# Autodesk Inventor assembly: Assembly1
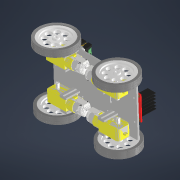
[picture p0: Inventor's stored thumbnail of the model, 180x180]
Saved by Autodesk Inventor 2021 (Build 250183000, 183)
## iProperties
Created: 2022-06-26
Part Number: Assembly1
Document SubType Name: Assembly
Designer: phand
Author: phand
## Documents named in this file (9)
- D:\Kien Phan\University\Training\Bluetooth controlling car\3D\Assembly1.iam
- D:\Kien Phan\University\Training\Bluetooth controlling car\3D\chassis.ipt
- D:\Kien Phan\University\Training\Bluetooth controlling car\3D\Ga motor 1.ipt
- D:\Kien Phan\University\Training\Bluetooth controlling car\3D\YG2900_step.ipt
- D:\Kien Phan\University\IAC Club\Animal Robot\Line follower robot\v4\rubber-wheel-65mm-1.snapshot.1\Whell - 65mm\Llanta.ipt
- D:\Kien Phan\University\IAC Club\Animal Robot\Line follower robot\v4\l298n-stepper-motor-driver-red-1.snapshot.3\L298N Stepper Motor Driver (Red).ipt
- D:\Kien Phan\University\Training\Bluetooth controlling car\3D\18650 battery holder part.ipt
- D:\Kien Phan\University\Training\Bluetooth controlling car\3D\mid chassis.ipt
- D:\Kien Phan\Inventor Library\Parts\Arduino Uno.ipt
## Components (21 placed, 8 different names)
1. chassis:1 — Mate:1, Mate:2, Mate:4, Mate:6, Mate:7, Mate:8, Mate:9, Mate:10, Mate:11, Mate:12, Mate:15, Mate:16, Mate:17, Mate:22, Mate:23, Mate:24, Mate:25, Mate:26, Mate:27, Mate:30, Mate:31, Mate:32, Mate:33, Mate:34, Mate:35, Mate:38, Mate:45, Mate:46, Mate:48, Mate:50, Mate:53, Mate:54, Mate:55
2. YG2900_step:4 — Mate:36, Mate:37, Mate:42
3. Ga motor 1:1 — Mate:1, Mate:2, Mate:4, Mate:6, Mate:21, Mate:38
4. Ga motor 1:2 — Mate:7, Mate:8, Mate:9, Mate:20
5. Ga motor 1:3 — Mate:15, Mate:16, Mate:17
6. Ga motor 1:4 — Mate:10, Mate:11, Mate:12, Mate:18, Mate:19
7. Ga motor 1:5 — Mate:32, Mate:33, Mate:34, Mate:36, Mate:37
8. Ga motor 1:6 — Mate:30, Mate:31, Mate:35, Mate:48
9. Ga motor 1:7 — Mate:25, Mate:26, Mate:27
10. Ga motor 1:8 — Mate:22, Mate:23, Mate:24, Mate:28, Mate:29
11. YG2900_step:5 — Mate:20, Mate:21, Mate:39
12. YG2900_step:6 — Mate:18, Mate:19, Mate:41
13. YG2900_step:7 — Mate:28, Mate:29, Mate:43
14. Llanta:1 — Mate:39
15. Llanta:3 — Mate:41
16. Llanta:4 — Mate:43
17. Llanta:5 — Mate:42
18. L298N Stepper Motor Driver (Red):1 — Mate:45, Mate:46
19. 18650 battery holder part:1 — Mate:52
20. mid chassis:1 — Mate:50, Mate:52
21. Arduino Uno:1 — Mate:53, Mate:54, Mate:55
## Relationships (46: Mate 46)
- Mate:1: chassis:1 ↔ Ga motor 1:1
- Mate:2: chassis:1 ↔ Ga motor 1:1
- Mate:4: chassis:1 ↔ Ga motor 1:1
- Mate:6: chassis:1 ↔ Ga motor 1:1
- Mate:7: chassis:1 ↔ Ga motor 1:2
- Mate:8: chassis:1 ↔ Ga motor 1:2
- Mate:9: chassis:1 ↔ Ga motor 1:2
- Mate:10: chassis:1 ↔ Ga motor 1:4
- Mate:11: chassis:1 ↔ Ga motor 1:4
- Mate:12: chassis:1 ↔ Ga motor 1:4
- Mate:15: chassis:1 ↔ Ga motor 1:3
- Mate:16: chassis:1 ↔ Ga motor 1:3
- Mate:17: chassis:1 ↔ Ga motor 1:3
- Mate:18: Ga motor 1:4 ↔ YG2900_step:6
- Mate:19: Ga motor 1:4 ↔ YG2900_step:6
- Mate:20: Ga motor 1:2 ↔ YG2900_step:5
- Mate:21: Ga motor 1:1 ↔ YG2900_step:5
- Mate:22: chassis:1 ↔ Ga motor 1:8
- Mate:23: chassis:1 ↔ Ga motor 1:8
- Mate:24: chassis:1 ↔ Ga motor 1:8
- Mate:25: chassis:1 ↔ Ga motor 1:7
- Mate:26: chassis:1 ↔ Ga motor 1:7
- Mate:27: chassis:1 ↔ Ga motor 1:7
- Mate:28: Ga motor 1:8 ↔ YG2900_step:7
- Mate:29: Ga motor 1:8 ↔ YG2900_step:7
- Mate:30: chassis:1 ↔ Ga motor 1:6
- Mate:31: chassis:1 ↔ Ga motor 1:6
- Mate:32: chassis:1 ↔ Ga motor 1:5
- Mate:33: chassis:1 ↔ Ga motor 1:5
- Mate:34: chassis:1 ↔ Ga motor 1:5
- Mate:35: chassis:1 ↔ Ga motor 1:6
- Mate:36: YG2900_step:4 ↔ Ga motor 1:5
- Mate:37: YG2900_step:4 ↔ Ga motor 1:5
- Mate:38: chassis:1 ↔ Ga motor 1:1
- Mate:39: YG2900_step:5 ↔ Llanta:1
- Mate:41: YG2900_step:6 ↔ Llanta:3
- Mate:42: YG2900_step:4 ↔ Llanta:5
- Mate:43: YG2900_step:7 ↔ Llanta:4
- Mate:45 (5 mm): chassis:1 ↔ L298N Stepper Motor Driver (Red):1
- Mate:46: chassis:1 ↔ L298N Stepper Motor Driver (Red):1
- Mate:48: chassis:1 ↔ Ga motor 1:6
- Mate:50 (5 mm): chassis:1 ↔ mid chassis:1
- Mate:52: 18650 battery holder part:1 ↔ mid chassis:1
- Mate:53: chassis:1 ↔ Arduino Uno:1
- Mate:54 (10 mm): chassis:1 ↔ Arduino Uno:1
- Mate:55: chassis:1 ↔ Arduino Uno:1
